# Autodesk Inventor assembly: A2017_T4_11
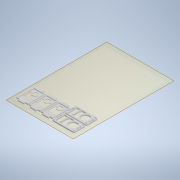
[picture p0: Inventor's stored thumbnail of the model, 180x180]
Saved by Autodesk Inventor 2020 (Build 240168000, 168)
## iProperties
Created: 2021-08-27
Part Number: A2017_T4_11
Document SubType Name: Assembly
Designer: Masato
Author: Masato
## Documents named in this file (4)
- C:\Inventor\SUSTAINA-OP\Cam\A2017_T4_11.iam
- C:\Inventor\SUSTAINA-OP\Cam\DisposableBoard.ipt
- C:\Inventor\SUSTAINA-OP\UpperBody\Trunk\Trunk_neck_frame.ipt
- C:\Inventor\SUSTAINA-OP\UpperBody\Trunk\Trunk_servo_bottom_frame.ipt
## Components (6 placed, 3 different names)
1. DisposableBoard:1 — メイト:2, メイト:1, フラッシュ:1, フラッシュ:2, メイト:8, フラッシュ:5, フラッシュ:6, メイト:10
2. Trunk_servo_bottom_frame:1 — メイト:8, フラッシュ:5, フラッシュ:6, フラッシュ:7
3. Trunk_servo_bottom_frame:2
4. Trunk_servo_bottom_frame:3 — メイト:11
5. Trunk_neck_frame:2 — メイト:10, フラッシュ:7, メイト:11
6. Trunk_neck_frame:3
## Component patterns: (3 elements, first: Trunk_servo_bottom_frame:1), (2 elements, first: Trunk_neck_frame:2)
## Relationships (10: Mate 5, Flush 5)
- メイト:2 [Mate]: DisposableBoard:1
- メイト:1 [Mate]: DisposableBoard:1
- フラッシュ:1 [Flush]: DisposableBoard:1
- フラッシュ:2 [Flush]: DisposableBoard:1
- メイト:8 [Mate]: DisposableBoard:1 ↔ Trunk_servo_bottom_frame:1
- フラッシュ:5 [Flush] (2 mm): DisposableBoard:1 ↔ Trunk_servo_bottom_frame:1
- フラッシュ:6 [Flush] (2 mm): DisposableBoard:1 ↔ Trunk_servo_bottom_frame:1
- メイト:10 [Mate]: DisposableBoard:1 ↔ Trunk_neck_frame:2
- フラッシュ:7 [Flush]: Trunk_servo_bottom_frame:1 ↔ Trunk_neck_frame:2
- メイト:11 [Mate] (2.5 mm): Trunk_servo_bottom_frame:3 ↔ Trunk_neck_frame:2
